# Autodesk Inventor assembly: demo
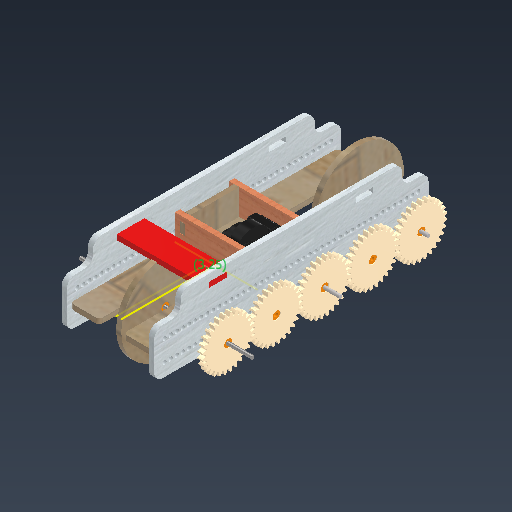
[picture p0: Inventor's stored thumbnail of the model, 512x512]
Saved by Autodesk Inventor 2025.3 (Build 293356000, 356)
## iProperties
Created: 2025-11-06
Part Number: demo
Document SubType Name: Assembly
Designer: 陳泓任
Author: 陳泓任
## Documents named in this file (15)
- C:\Users\Ou918\3D-model-temp\introduction to mechanical engineering(1)\version_6\demo.iam
- C:\Users\Ou918\3D-model-temp\introduction to mechanical engineering(1)\發條組合\發條組合.iam
- C:\Users\Ou918\3D-model-temp\introduction to mechanical engineering(1)\version_6\baffle_back_short.ipt
- C:\Users\Ou918\3D-model-temp\introduction to mechanical engineering(1)\version_6\baffle_front_short.ipt
- C:\Users\Ou918\3D-model-temp\introduction to mechanical engineering(1)\version_6\beam.ipt
- C:\Users\Ou918\3D-model-temp\introduction to mechanical engineering(1)\version_5\support_edited.ipt
- C:\Users\Ou918\3D-model-temp\introduction to mechanical engineering(1)\version_5\bolt.ipt
- C:\Users\Ou918\3D-model-temp\introduction to mechanical engineering(1)\sleeve.ipt
- C:\Users\Ou918\3D-model-temp\introduction to mechanical engineering(1)\big gear(with sleeve).iam
- C:\Users\Ou918\3D-model-temp\introduction to mechanical engineering(1)\51mm wheel(with sleeve).iam
- C:\Users\Ou918\3D-model-temp\introduction to mechanical engineering(1)\100mm rod.ipt
- C:\Users\Ou918\3D-model-temp\introduction to mechanical engineering(1)\80mm rod.ipt
- C:\Users\Ou918\3D-model-temp\introduction to mechanical engineering(1)\small gear(with sleeve).iam
- C:\Users\Ou918\3D-model-temp\introduction to mechanical engineering(1)\version_6\main_frame.ipt
- C:\Users\Ou918\3D-model-temp\introduction to mechanical engineering(1)\version_6\side_frame(minus 7).ipt
## Components (23 placed, 14 different names)
1. main_frame:1 — 貼合:48, 貼合:49, 貼合:50, 齊平:7, 貼合:51, 貼合:55, 角度:2, 齊平:8, 貼合:60, 貼合:61, 貼合:63
2. 發條組合:1 [sub-assembly] — 貼合:16, 貼合:31, 貼合:32, 齊平:7, 貼合:55, 貼合:70
3. baffle_back_short:1 — 貼合:20, 貼合:26, 貼合:53, 貼合:54, 貼合:56
4. baffle_front_short:1 — 貼合:16, 貼合:23, 貼合:25, 貼合:49, 貼合:51, 貼合:52
5. beam:1 — 貼合:71, 貼合:72, 貼合:73
6. beam:2 — 貼合:64, 貼合:65, 貼合:66, 貼合:67, 貼合:68, 貼合:69
7. support_edited:1 — 貼合:20, 貼合:23, 貼合:27, 貼合:29, 貼合:48, 貼合:50, 貼合:52, 貼合:53, 貼合:54
8. support_edited:2 — 貼合:25, 貼合:26, 貼合:28, 貼合:56
9. bolt:1 — 貼合:27, 貼合:28, 貼合:29
10. sleeve:1 — 貼合:31, 貼合:33
11. big gear(with sleeve):1 [sub-assembly] — 貼合:32, 貼合:33, 齊平:2, 齊平:5
12. 51mm wheel(with sleeve):1 [sub-assembly] — with_wheel
13. 51mm wheel(with sleeve):3 [sub-assembly] — 貼合:45
14. 100mm rod:1 — 貼合:38, 貼合:60, with_wheel, 貼合:62, 貼合:75, 貼合:76
15. sleeve:2 — 貼合:38
16. big gear(with sleeve):3 [sub-assembly] — 齊平:1
17. big gear(with sleeve):5 [sub-assembly] — 齊平:4, 齊平:5
18. big gear(with sleeve):6 [sub-assembly] — 齊平:4, 貼合:43
19. 80mm rod:1 — 貼合:43, 貼合:45, 貼合:61
20. big gear(with sleeve):4 [sub-assembly] — 齊平:1, 齊平:2, 貼合:76
21. small gear(with sleeve):1 [sub-assembly] — 貼合:74
22. side_frame(minus 7):1 — 貼合:66, 貼合:67, 貼合:68, 貼合:70, 齊平:9
23. side_frame(minus 7):2 — 貼合:62, 貼合:63, 貼合:64, 貼合:65, 貼合:69, 齊平:9, 角度:3, 貼合:71, 貼合:72, 貼合:73, 貼合:74, 貼合:75
## Relationships (50: Mate 41, Flush 7, Angle 2)
- 貼合:16 [Mate]: 發條組合:1 ↔ baffle_front_short:1
- 貼合:20 [Mate]: baffle_back_short:1 ↔ support_edited:1
- 貼合:23 [Mate]: baffle_front_short:1 ↔ support_edited:1
- 貼合:25 [Mate]: baffle_front_short:1 ↔ support_edited:2
- 貼合:26 [Mate]: baffle_back_short:1 ↔ support_edited:2
- 貼合:27 [Mate]: support_edited:1 ↔ bolt:1
- 貼合:28 [Mate]: support_edited:2 ↔ bolt:1
- 貼合:29 [Mate]: support_edited:1 ↔ bolt:1
- 貼合:31 [Mate]: 發條組合:1 ↔ sleeve:1
- 貼合:32 [Mate]: 發條組合:1 ↔ big gear(with sleeve):1
- 貼合:33 [Mate]: sleeve:1 ↔ big gear(with sleeve):1
- 貼合:38 [Mate]: 100mm rod:1 ↔ sleeve:2
- 貼合:60 [Mate]: main_frame:1 ↔ 100mm rod:1
- with_wheel [Mate]: 51mm wheel(with sleeve):1 ↔ 100mm rod:1
- 齊平:1 [Flush]: big gear(with sleeve):3 ↔ big gear(with sleeve):4
- 齊平:2 [Flush]: big gear(with sleeve):1 ↔ big gear(with sleeve):4
- 齊平:4 [Flush]: big gear(with sleeve):5 ↔ big gear(with sleeve):6
- 齊平:5 [Flush]: big gear(with sleeve):1 ↔ big gear(with sleeve):5
- 貼合:43 [Mate]: big gear(with sleeve):6 ↔ 80mm rod:1
- 貼合:45 [Mate]: 51mm wheel(with sleeve):3 ↔ 80mm rod:1
- 貼合:48 [Mate]: main_frame:1 ↔ support_edited:1
- 貼合:49 [Mate]: main_frame:1 ↔ baffle_front_short:1
- 貼合:50 [Mate]: main_frame:1 ↔ support_edited:1
- 齊平:7 [Flush] (-6.75 mm): main_frame:1 ↔ 發條組合:1
- 貼合:51 [Mate]: main_frame:1 ↔ baffle_front_short:1
- 貼合:52 [Mate]: baffle_front_short:1 ↔ support_edited:1
- 貼合:53 [Mate]: baffle_back_short:1 ↔ support_edited:1
- 貼合:54 [Mate]: baffle_back_short:1 ↔ support_edited:1
- 貼合:55 [Mate]: main_frame:1 ↔ 發條組合:1
- 貼合:56 [Mate]: baffle_back_short:1 ↔ support_edited:2
- 角度:2 [Angle] (0 deg): main_frame:1
- 齊平:8 [Flush]: main_frame:1
- 貼合:61 [Mate]: main_frame:1 ↔ 80mm rod:1
- 貼合:62 [Mate]: 100mm rod:1 ↔ side_frame(minus 7):2
- 貼合:63 [Mate]: main_frame:1 ↔ side_frame(minus 7):2
- 貼合:64 [Mate]: beam:2 ↔ side_frame(minus 7):2
- 貼合:65 [Mate]: beam:2 ↔ side_frame(minus 7):2
- 貼合:66 [Mate]: beam:2 ↔ side_frame(minus 7):1
- 貼合:67 [Mate]: beam:2 ↔ side_frame(minus 7):1
- 貼合:68 [Mate]: beam:2 ↔ side_frame(minus 7):1
- 貼合:69 [Mate]: beam:2 ↔ side_frame(minus 7):2
- 貼合:70 [Mate]: 發條組合:1 ↔ side_frame(minus 7):1
- 齊平:9 [Flush]: side_frame(minus 7):1 ↔ side_frame(minus 7):2
- 角度:3 [Angle] (0 deg): side_frame(minus 7):2
- 貼合:71 [Mate]: beam:1 ↔ side_frame(minus 7):2
- 貼合:72 [Mate]: beam:1 ↔ side_frame(minus 7):2
- 貼合:73 [Mate]: beam:1 ↔ side_frame(minus 7):2
- 貼合:74 [Mate]: small gear(with sleeve):1 ↔ side_frame(minus 7):2
- 貼合:75 [Mate]: 100mm rod:1 ↔ side_frame(minus 7):2
- 貼合:76 [Mate]: 100mm rod:1 ↔ big gear(with sleeve):4
